# Autodesk Inventor assembly: Saw set up
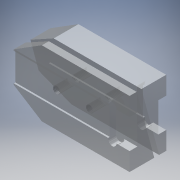
[picture p0: Inventor's stored thumbnail of the model, 180x180]
Saved by Autodesk Inventor 2018 (Build 220112000, 112)
## iProperties
Created: 2018-12-10
Part Number: Saw set up
Project: =<Part Number>
Document SubType Name: Assembly
Designer: S.O.
Author: S.O.
## Documents named in this file (2)
- R:\CAD\~Aquafil~\7407 - 456 Slant Blades-72 Flat Blades (Standard Size)\CAD\Saw set up.iam
- R:\CAD\~Aquafil~\7407 - 456 Slant Blades-72 Flat Blades (Standard Size)\CAD\DHC-1500-FF-02-003.ipt
## Components (2 placed, 1 different names)
1. DHC-1500-FF-02-003:1 — Flush:1, Flush:2, Mate:1
2. DHC-1500-FF-02-003:2 — Flush:1, Flush:2, Mate:1
## Relationships (3: Flush 2, Mate 1)
- Flush:1: DHC-1500-FF-02-003:1 ↔ DHC-1500-FF-02-003:2
- Flush:2: DHC-1500-FF-02-003:1 ↔ DHC-1500-FF-02-003:2
- Mate:1 (-44.45 mm): DHC-1500-FF-02-003:1 ↔ DHC-1500-FF-02-003:2
